# Autodesk Inventor assembly: fourBar
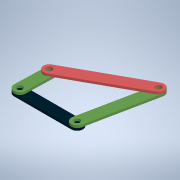
[picture p0: Inventor's stored thumbnail of the model, 180x180]
Saved by Autodesk Inventor 2020.1 (Build 241239000, 239)
## iProperties
Created: 2019-08-08
Part Number: fourBar
Document SubType Name: Assembly
Designer: sshel
Author: sshel
## Documents named in this file (5)
- D:\Desktop 2019\MS, Phd\Sem7- 2018 Fall (RA, 3research)\N-Bar analysis\Inventor Planar\fourBar.iam
- D:\Desktop 2019\MS, Phd\Sem7- 2018 Fall (RA, 3research)\N-Bar analysis\Inventor Planar\Base.ipt
- D:\Desktop 2019\MS, Phd\Sem7- 2018 Fall (RA, 3research)\N-Bar analysis\Inventor Planar\Input.ipt
- D:\Desktop 2019\MS, Phd\Sem7- 2018 Fall (RA, 3research)\N-Bar analysis\Inventor Planar\Output.ipt
- D:\Desktop 2019\MS, Phd\Sem7- 2018 Fall (RA, 3research)\N-Bar analysis\Inventor Planar\Coupler.ipt
## Components (4 placed, 4 different names)
1. Base:1 — InpPl, InpPt, OutPl, OutPt
2. Input:1 — InpPl, InpPt, MPInp
3. Output:1 — OutPl, OutPt, MPOut
4. Coupler:1 — MPInp, MPOut
## Relationships (6: Mate 6)
- InpPl [Mate]: Base:1 ↔ Input:1
- InpPt [Mate]: Base:1 ↔ Input:1
- OutPl [Mate]: Base:1 ↔ Output:1
- OutPt [Mate]: Base:1 ↔ Output:1
- MPInp [Mate]: Input:1 ↔ Coupler:1
- MPOut [Mate]: Output:1 ↔ Coupler:1
